# Autodesk Inventor assembly: Marker Changer
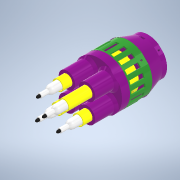
[picture p0: Inventor's stored thumbnail of the model, 180x180]
Saved by Autodesk Inventor 2022.2 (Build 262287000, 287)
## iProperties
Created: 2022-02-09
Part Number: Marker Changer
Document SubType Name: Assembly
Designer: smiku
Author: smiku
## Documents named in this file (10)
- C:\Users\smiku\3D Objects\GrabCAD\AACC Mechatonics Capstone\Marker Changer\Marker Changer.iam
- C:\Users\smiku\3D Objects\GrabCAD\AACC Mechatonics Capstone\Marker Changer\Cam Barrel Plate.ipt
- C:\Users\smiku\3D Objects\GrabCAD\AACC Mechatonics Capstone\Marker Changer\Single Cam Plate.ipt
- C:\Users\smiku\3D Objects\GrabCAD\AACC Mechatonics Capstone\Interface\Servo\Servo Hub.ipt
- C:\Users\smiku\3D Objects\GrabCAD\AACC Mechatonics Capstone\Interface\Servo\DS3225mg Servo.ipt
- C:\Users\smiku\3D Objects\GrabCAD\AACC Mechatonics Capstone\Interface\Interface Block.ipt
- C:\Users\smiku\3D Objects\GrabCAD\AACC Mechatonics Capstone\Marker Changer\Case.ipt
- C:\Users\smiku\3D Objects\GrabCAD\AACC Mechatonics Capstone\Marker Changer\Hoop.ipt
- C:\Users\smiku\3D Objects\GrabCAD\AACC Mechatonics Capstone\Marker Changer\Static Marker Barrel.ipt
- C:\Users\smiku\3D Objects\GrabCAD\AACC Mechatonics Capstone\Interface\Marker\Expo Marker Bullet Point.ipt
## Components (15 placed, 9 different names)
1. Interface Block:1 — Rigid:7
2. Case:1 — Rigid:6, Rigid:7, Rigid:8
3. DS3225mg Servo:1 — Rotational:2, Rigid:6
4. Hoop:1 — Rigid:5, Rigid:8
5. Servo Hub:1 — Rigid:1, Rotational:2
6. Single Cam Plate:1 — Rigid:1
7. Cam Barrel Plate:1 — Cylindrical:1, Cylindrical:2, Cylindrical:3, Cylindrical:4, Rigid:5
8. Static Marker Barrel:1 — Cylindrical:1, Rigid:10
9. Static Marker Barrel:2 — Cylindrical:2, Rigid:11
10. Static Marker Barrel:3 — Cylindrical:3, Rigid:9
11. Static Marker Barrel:4 — Cylindrical:4, Rigid:12
12. Expo Marker Bullet Point:1 — Rigid:9
13. Expo Marker Bullet Point:2 — Rigid:10
14. Expo Marker Bullet Point:3 — Rigid:11
15. Expo Marker Bullet Point:4 — Rigid:12
## Relationships (14: WeldJoint 9, CylindricalJoint 4, RevoluteJoint 1)
- Cylindrical:1: Cam Barrel Plate:1 ↔ Static Marker Barrel:1
- Cylindrical:2: Cam Barrel Plate:1 ↔ Static Marker Barrel:2
- Cylindrical:3: Cam Barrel Plate:1 ↔ Static Marker Barrel:3
- Cylindrical:4: Cam Barrel Plate:1 ↔ Static Marker Barrel:4
- Rigid:1 [WeldJoint]: Servo Hub:1 ↔ Single Cam Plate:1
- Rotational:2 [RevoluteJoint]: DS3225mg Servo:1 ↔ Servo Hub:1
- Rigid:5 [WeldJoint]: Hoop:1 ↔ Cam Barrel Plate:1
- Rigid:6 [WeldJoint]: Case:1 ↔ DS3225mg Servo:1
- Rigid:7 [WeldJoint]: Interface Block:1 ↔ Case:1
- Rigid:8 [WeldJoint]: Case:1 ↔ Hoop:1
- Rigid:9 [WeldJoint]: Static Marker Barrel:3 ↔ Expo Marker Bullet Point:1
- Rigid:10 [WeldJoint]: Static Marker Barrel:1 ↔ Expo Marker Bullet Point:2
- Rigid:11 [WeldJoint]: Static Marker Barrel:2 ↔ Expo Marker Bullet Point:3
- Rigid:12 [WeldJoint]: Static Marker Barrel:4 ↔ Expo Marker Bullet Point:4
